# Autodesk Inventor assembly: waterjet assembly version
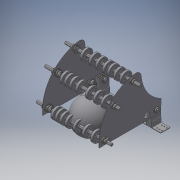
[picture p0: Inventor's stored thumbnail of the model, 180x180]
Saved by Autodesk Inventor 2018 (Build 220112000, 112)
## iProperties
Created: 2020-01-24
Part Number: waterjet assembly version
Document SubType Name: Assembly
Designer: s-2513225
Author: s-2513225
## Documents named in this file (12)
- \\studenthome\students\S-2513225\GitHub\2020CAD\Over bumper intake\Assembly\waterjet assembly version.iam
- \\studenthome\students\S-2513225\GitHub\2020CAD\Over bumper intake\Parts\waterjet wall.ipt
- \\studenthome\students\S-2513225\GitHub\2020CAD\Over bumper intake\Parts\0_500_Hex_ID_x_1_125_OD_x_0_313_WD_Flanged_Bearing_v2_217-3875.ipt
- \\studenthome\students\S-2513225\GitHub\2020CAD\Over bumper intake\Parts\hex shaft 1.ipt
- \\studenthome\students\S-2513225\GitHub\2020CAD\Over bumper intake\Parts\ball mock up.ipt
- \\studenthome\students\S-2513225\GitHub\2020CAD\Over bumper intake\Parts\banebots 400 - 2 3-8 replacement.ipt
- \\studenthome\students\S-2513225\GitHub\2020CAD\Over bumper intake\Parts\anchor point.ipt
- \\studenthome\students\S-2513225\GitHub\2020CAD\Over bumper intake\Parts\hex 2.ipt
- \\studenthome\students\S-2513225\GitHub\2020CAD\Over bumper intake\Parts\2in bracket.ipt
- \\studenthome\students\S-2513225\GitHub\2020CAD\Over bumper intake\Parts\VersaPlanetary_v2_Single_Stage_10_1_with_775_Series.iam
- \\studenthome\students\S-2513225\GitHub\2020CAD\Over bumper intake\Parts\_16t_Aluminum_Hub_Sprocket_25_Chain_1_2_Hex_Bore_217-2642.ipt
- \\studenthome\students\S-2513225\GitHub\2020CAD\Over bumper intake\Parts\Clamping_Shaft_Collar_-_1_2_Hex_ID_217-2737.ipt
## Components (70 placed, 11 different names)
1. waterjet wall:1 — Mate:2, Mate:4, Mate:5, Mate:6, Mate:7, Mate:8, Mate:9, Mate:26, Mate:79, Mate:90, Mate:91, Mate:97, Mate:108, Mate:109, Flush:11, Flush:12, Symmetry:1
2. waterjet wall:2 — Mate:16, Mate:17, Mate:18, Mate:19, Mate:20, Mate:21, Mate:22, Mate:26, Mate:88, Mate:89, Mate:99, Symmetry:1, Flush:13
3. 0_500_Hex_ID_x_1_125_OD_x_0_313_WD_Flanged_Bearing_v2_217-3875:1 — Mate:5, Mate:7, Mate:10, Mate:15
4. 0_500_Hex_ID_x_1_125_OD_x_0_313_WD_Flanged_Bearing_v2_217-3875:2 — Mate:6, Mate:9, Mate:12, Mate:14
5. 0_500_Hex_ID_x_1_125_OD_x_0_313_WD_Flanged_Bearing_v2_217-3875:3 — Mate:4, Mate:8, Mate:11, Mate:13
6. 0_500_Hex_ID_x_1_125_OD_x_0_313_WD_Flanged_Bearing_v2_217-3875:4 — Mate:19, Mate:21, Mate:24
7. 0_500_Hex_ID_x_1_125_OD_x_0_313_WD_Flanged_Bearing_v2_217-3875:5 — Mate:18, Mate:20, Mate:23, Mate:25
8. 0_500_Hex_ID_x_1_125_OD_x_0_313_WD_Flanged_Bearing_v2_217-3875:6 — Mate:17, Mate:22
9. hex shaft 1:1 — Mate:12, Mate:14, Mate:23, Mate:25, Mate:37, Mate:53, Mate:68, Mate:72, Mate:73, Mate:74, Mate:75, Mate:76, Mate:77, Mate:78, Mate:104, Mate:105, Mate:106, Mate:107, Flush:11, Mate:118, Mate:119, Mate:122, Mate:123, Mate:138, Mate:139, Mate:149
10. hex shaft 1:2 — Mate:10, Mate:15, Mate:27, Mate:28, Mate:29, Mate:30, Mate:39, Mate:42, Mate:43, Mate:44, Mate:45, Mate:46, Mate:61, Mate:62, Mate:63, Mate:64, Mate:130, Mate:131, Mate:132, Mate:133, Mate:134, Mate:135, Mate:136, Mate:147
11. hex shaft 1:3 — Mate:11, Mate:13, Mate:24, Mate:31, Mate:32, Mate:33, Mate:34, Mate:40, Mate:47, Mate:48, Mate:49, Mate:50, Mate:51, Mate:65, Mate:66, Mate:69, Mate:70, Mate:124, Mate:125, Mate:126, Mate:127, Mate:128, Mate:129, Mate:137, Mate:148
12. ball mock up:1
13. banebots 400 - 2 3-8 replacement:1 — Mate:27, Mate:42
14. banebots 400 - 2 3-8 replacement:2 — Mate:30, Mate:43
15. banebots 400 - 2 3-8 replacement:3 — Mate:31, Mate:50
16. banebots 400 - 2 3-8 replacement:4 — Mate:29, Mate:44
17. banebots 400 - 2 3-8 replacement:5 — Mate:40, Mate:51
18. banebots 400 - 2 3-8 replacement:6 — Mate:28, Mate:46
19. banebots 400 - 2 3-8 replacement:7 — Mate:34, Mate:47
20. banebots 400 - 2 3-8 replacement:8 — Mate:32, Mate:48
21. banebots 400 - 2 3-8 replacement:9 — Mate:39, Mate:45
22. banebots 400 - 2 3-8 replacement:10 — Mate:73, Mate:78
23. banebots 400 - 2 3-8 replacement:11 — Mate:37, Mate:53
24. banebots 400 - 2 3-8 replacement:12 — Mate:75, Mate:76
25. banebots 400 - 2 3-8 replacement:13 — Mate:105, Mate:106
26. banebots 400 - 2 3-8 replacement:14 — Mate:33, Mate:49
27. banebots 400 - 2 3-8 replacement:15 — Mate:104, Mate:107
28. banebots 400 - 2 3-8 replacement:16 — Mate:61, Mate:63
29. banebots 400 - 2 3-8 replacement:17 — Mate:62, Mate:64
30. banebots 400 - 2 3-8 replacement:18 — Mate:66, Mate:70
31. banebots 400 - 2 3-8 replacement:19 — Mate:65, Mate:69
32. banebots 400 - 2 3-8 replacement:20 — Mate:74, Mate:77
33. banebots 400 - 2 3-8 replacement:21 — Mate:68, Mate:72
34. anchor point:1 — Mate:80, Mate:81, Mate:82, Mate:83, Mate:97, Flush:5, Mate:101, Flush:6, Flush:9, Flush:10, Mate:103
35. anchor point:2 — Mate:84, Mate:85, Mate:86, Mate:87, Mate:99, Mate:100, Flush:3, Flush:4, Mate:102, Flush:7, Flush:8
36. 0_500_Hex_ID_x_1_125_OD_x_0_313_WD_Flanged_Bearing_v2_217-3875:7 — Mate:80, Mate:81, Mate:96
37. 0_500_Hex_ID_x_1_125_OD_x_0_313_WD_Flanged_Bearing_v2_217-3875:8 — Mate:82, Mate:83
38. 0_500_Hex_ID_x_1_125_OD_x_0_313_WD_Flanged_Bearing_v2_217-3875:9 — Mate:84, Mate:85, Mate:98
39. 0_500_Hex_ID_x_1_125_OD_x_0_313_WD_Flanged_Bearing_v2_217-3875:10 — Mate:86, Mate:87
40. 0_500_Hex_ID_x_1_125_OD_x_0_313_WD_Flanged_Bearing_v2_217-3875:11 — Mate:88, Mate:89, Mate:92, Mate:94
41. 0_500_Hex_ID_x_1_125_OD_x_0_313_WD_Flanged_Bearing_v2_217-3875:12 — Mate:90, Mate:91, Mate:93, Mate:95
42. hex 2:1 — Mate:93, Mate:95, Mate:96, Mate:110, Mate:111, Mate:112, Mate:113
43. hex 2:2 — Mate:92, Mate:94, Mate:98, Mate:114, Mate:115, Mate:116, Mate:117
44. 2in bracket:1 — Flush:5, Mate:101, Flush:6, Flush:12
45. 2in bracket:2 — Mate:100, Flush:3, Flush:4, Flush:13
46. 2in bracket:3 — Mate:102, Flush:7, Flush:8
47. 2in bracket:4 — Flush:9, Flush:10, Mate:103
48. VersaPlanetary_v2_Single_Stage_10_1_with_775_Series:1 [sub-assembly] — Mate:142, Mate:143, Mate:144, Mate:145, Mate:146
49. 0_500_Hex_ID_x_1_125_OD_x_0_313_WD_Flanged_Bearing_v2_217-3875:13 — Mate:108, Mate:109, Mate:144
50. _16t_Aluminum_Hub_Sprocket_25_Chain_1_2_Hex_Bore_217-2642:1 — Mate:130, Mate:131
51. _16t_Aluminum_Hub_Sprocket_25_Chain_1_2_Hex_Bore_217-2642:2 — Mate:118, Mate:119
52. _16t_Aluminum_Hub_Sprocket_25_Chain_1_2_Hex_Bore_217-2642:4 — Mate:124, Mate:125
53. Clamping_Shaft_Collar_-_1_2_Hex_ID_217-2737:1 — Mate:122, Mate:123
54. Clamping_Shaft_Collar_-_1_2_Hex_ID_217-2737:2 — Mate:128, Mate:129
55. Clamping_Shaft_Collar_-_1_2_Hex_ID_217-2737:3 — Mate:134, Mate:135
56. Clamping_Shaft_Collar_-_1_2_Hex_ID_217-2737:4 — Mate:138, Mate:139
57. Clamping_Shaft_Collar_-_1_2_Hex_ID_217-2737:5 — Mate:137
58. Clamping_Shaft_Collar_-_1_2_Hex_ID_217-2737:6 — Mate:136
59. Clamping_Shaft_Collar_-_1_2_Hex_ID_217-2737:7 — Mate:114, Mate:115
60. Clamping_Shaft_Collar_-_1_2_Hex_ID_217-2737:8 — Mate:116, Mate:117
61. Clamping_Shaft_Collar_-_1_2_Hex_ID_217-2737:9 — Mate:110, Mate:111
62. Clamping_Shaft_Collar_-_1_2_Hex_ID_217-2737:10 — Mate:112, Mate:113
63. Clamping_Shaft_Collar_-_1_2_Hex_ID_217-2737:11 — Mate:147
64. _16t_Aluminum_Hub_Sprocket_25_Chain_1_2_Hex_Bore_217-2642:5 — Mate:126, Mate:127
65. _16t_Aluminum_Hub_Sprocket_25_Chain_1_2_Hex_Bore_217-2642:6 — Mate:132, Mate:133
66. _16t_Aluminum_Hub_Sprocket_25_Chain_1_2_Hex_Bore_217-2642:7
67. Clamping_Shaft_Collar_-_1_2_Hex_ID_217-2737:12 — Mate:142, Mate:143
68. _16t_Aluminum_Hub_Sprocket_25_Chain_1_2_Hex_Bore_217-2642:8 — Mate:145, Mate:146
69. Clamping_Shaft_Collar_-_1_2_Hex_ID_217-2737:13 — Mate:148
70. Clamping_Shaft_Collar_-_1_2_Hex_ID_217-2737:15 — Mate:149
## Relationships (141: Mate 129, Flush 11, Symmetry 1)
- Mate:2: waterjet wall:1
- Mate:4: waterjet wall:1 ↔ 0_500_Hex_ID_x_1_125_OD_x_0_313_WD_Flanged_Bearing_v2_217-3875:3
- Mate:5: waterjet wall:1 ↔ 0_500_Hex_ID_x_1_125_OD_x_0_313_WD_Flanged_Bearing_v2_217-3875:1
- Mate:6: waterjet wall:1 ↔ 0_500_Hex_ID_x_1_125_OD_x_0_313_WD_Flanged_Bearing_v2_217-3875:2
- Mate:7: waterjet wall:1 ↔ 0_500_Hex_ID_x_1_125_OD_x_0_313_WD_Flanged_Bearing_v2_217-3875:1
- Mate:8: waterjet wall:1 ↔ 0_500_Hex_ID_x_1_125_OD_x_0_313_WD_Flanged_Bearing_v2_217-3875:3
- Mate:9: waterjet wall:1 ↔ 0_500_Hex_ID_x_1_125_OD_x_0_313_WD_Flanged_Bearing_v2_217-3875:2
- Mate:10: 0_500_Hex_ID_x_1_125_OD_x_0_313_WD_Flanged_Bearing_v2_217-3875:1 ↔ hex shaft 1:2
- Mate:11: 0_500_Hex_ID_x_1_125_OD_x_0_313_WD_Flanged_Bearing_v2_217-3875:3 ↔ hex shaft 1:3
- Mate:12: 0_500_Hex_ID_x_1_125_OD_x_0_313_WD_Flanged_Bearing_v2_217-3875:2 ↔ hex shaft 1:1
- Mate:13: 0_500_Hex_ID_x_1_125_OD_x_0_313_WD_Flanged_Bearing_v2_217-3875:3 ↔ hex shaft 1:3
- Mate:14: 0_500_Hex_ID_x_1_125_OD_x_0_313_WD_Flanged_Bearing_v2_217-3875:2 ↔ hex shaft 1:1
- Mate:15: 0_500_Hex_ID_x_1_125_OD_x_0_313_WD_Flanged_Bearing_v2_217-3875:1 ↔ hex shaft 1:2
- Mate:16: waterjet wall:2
- Mate:17: waterjet wall:2 ↔ 0_500_Hex_ID_x_1_125_OD_x_0_313_WD_Flanged_Bearing_v2_217-3875:6
- Mate:18: waterjet wall:2 ↔ 0_500_Hex_ID_x_1_125_OD_x_0_313_WD_Flanged_Bearing_v2_217-3875:5
- Mate:19: waterjet wall:2 ↔ 0_500_Hex_ID_x_1_125_OD_x_0_313_WD_Flanged_Bearing_v2_217-3875:4
- Mate:20: waterjet wall:2 ↔ 0_500_Hex_ID_x_1_125_OD_x_0_313_WD_Flanged_Bearing_v2_217-3875:5
- Mate:21: waterjet wall:2 ↔ 0_500_Hex_ID_x_1_125_OD_x_0_313_WD_Flanged_Bearing_v2_217-3875:4
- Mate:22: waterjet wall:2 ↔ 0_500_Hex_ID_x_1_125_OD_x_0_313_WD_Flanged_Bearing_v2_217-3875:6
- Mate:23: 0_500_Hex_ID_x_1_125_OD_x_0_313_WD_Flanged_Bearing_v2_217-3875:5 ↔ hex shaft 1:1
- Mate:24: 0_500_Hex_ID_x_1_125_OD_x_0_313_WD_Flanged_Bearing_v2_217-3875:4 ↔ hex shaft 1:3
- Mate:25: 0_500_Hex_ID_x_1_125_OD_x_0_313_WD_Flanged_Bearing_v2_217-3875:5 ↔ hex shaft 1:1
- Mate:26 (304.8 mm): waterjet wall:1 ↔ waterjet wall:2
- Mate:27: hex shaft 1:2 ↔ banebots 400 - 2 3-8 replacement:1
- Mate:28: hex shaft 1:2 ↔ banebots 400 - 2 3-8 replacement:6
- Mate:29: hex shaft 1:2 ↔ banebots 400 - 2 3-8 replacement:4
- Mate:30: hex shaft 1:2 ↔ banebots 400 - 2 3-8 replacement:2
- Mate:31: hex shaft 1:3 ↔ banebots 400 - 2 3-8 replacement:3
- Mate:32: hex shaft 1:3 ↔ banebots 400 - 2 3-8 replacement:8
- Mate:33: hex shaft 1:3 ↔ banebots 400 - 2 3-8 replacement:14
- Mate:34: hex shaft 1:3 ↔ banebots 400 - 2 3-8 replacement:7
- Mate:37: hex shaft 1:1 ↔ banebots 400 - 2 3-8 replacement:11
- Mate:39: hex shaft 1:2 ↔ banebots 400 - 2 3-8 replacement:9
- Mate:40: hex shaft 1:3 ↔ banebots 400 - 2 3-8 replacement:5
- Mate:42: hex shaft 1:2 ↔ banebots 400 - 2 3-8 replacement:1
- Mate:43: hex shaft 1:2 ↔ banebots 400 - 2 3-8 replacement:2
- Mate:44: hex shaft 1:2 ↔ banebots 400 - 2 3-8 replacement:4
- Mate:45: hex shaft 1:2 ↔ banebots 400 - 2 3-8 replacement:9
- Mate:46: hex shaft 1:2 ↔ banebots 400 - 2 3-8 replacement:6
- Mate:47: hex shaft 1:3 ↔ banebots 400 - 2 3-8 replacement:7
- Mate:48: hex shaft 1:3 ↔ banebots 400 - 2 3-8 replacement:8
- Mate:49: hex shaft 1:3 ↔ banebots 400 - 2 3-8 replacement:14
- Mate:50: hex shaft 1:3 ↔ banebots 400 - 2 3-8 replacement:3
- Mate:51: hex shaft 1:3 ↔ banebots 400 - 2 3-8 replacement:5
- Mate:53: hex shaft 1:1 ↔ banebots 400 - 2 3-8 replacement:11
- Mate:61: hex shaft 1:2 ↔ banebots 400 - 2 3-8 replacement:16
- Mate:62: hex shaft 1:2 ↔ banebots 400 - 2 3-8 replacement:17
- Mate:63: hex shaft 1:2 ↔ banebots 400 - 2 3-8 replacement:16
- Mate:64: hex shaft 1:2 ↔ banebots 400 - 2 3-8 replacement:17
- Mate:65: hex shaft 1:3 ↔ banebots 400 - 2 3-8 replacement:19
- Mate:66: hex shaft 1:3 ↔ banebots 400 - 2 3-8 replacement:18
- Mate:68: hex shaft 1:1 ↔ banebots 400 - 2 3-8 replacement:21
- Mate:69: hex shaft 1:3 ↔ banebots 400 - 2 3-8 replacement:19
- Mate:70: hex shaft 1:3 ↔ banebots 400 - 2 3-8 replacement:18
- Mate:72: hex shaft 1:1 ↔ banebots 400 - 2 3-8 replacement:21
- Mate:73: hex shaft 1:1 ↔ banebots 400 - 2 3-8 replacement:10
- Mate:74: hex shaft 1:1 ↔ banebots 400 - 2 3-8 replacement:20
- Mate:75: hex shaft 1:1 ↔ banebots 400 - 2 3-8 replacement:12
- Mate:76: hex shaft 1:1 ↔ banebots 400 - 2 3-8 replacement:12
- Mate:77: hex shaft 1:1 ↔ banebots 400 - 2 3-8 replacement:20
- Mate:78: hex shaft 1:1 ↔ banebots 400 - 2 3-8 replacement:10
- Mate:79: waterjet wall:1
- Mate:80: anchor point:1 ↔ 0_500_Hex_ID_x_1_125_OD_x_0_313_WD_Flanged_Bearing_v2_217-3875:7
- Mate:81: anchor point:1 ↔ 0_500_Hex_ID_x_1_125_OD_x_0_313_WD_Flanged_Bearing_v2_217-3875:7
- Mate:82: anchor point:1 ↔ 0_500_Hex_ID_x_1_125_OD_x_0_313_WD_Flanged_Bearing_v2_217-3875:8
- Mate:83: anchor point:1 ↔ 0_500_Hex_ID_x_1_125_OD_x_0_313_WD_Flanged_Bearing_v2_217-3875:8
- Mate:84: anchor point:2 ↔ 0_500_Hex_ID_x_1_125_OD_x_0_313_WD_Flanged_Bearing_v2_217-3875:9
- Mate:85: anchor point:2 ↔ 0_500_Hex_ID_x_1_125_OD_x_0_313_WD_Flanged_Bearing_v2_217-3875:9
- Mate:86: anchor point:2 ↔ 0_500_Hex_ID_x_1_125_OD_x_0_313_WD_Flanged_Bearing_v2_217-3875:10
- Mate:87: anchor point:2 ↔ 0_500_Hex_ID_x_1_125_OD_x_0_313_WD_Flanged_Bearing_v2_217-3875:10
- Mate:88: waterjet wall:2 ↔ 0_500_Hex_ID_x_1_125_OD_x_0_313_WD_Flanged_Bearing_v2_217-3875:11
- Mate:89: waterjet wall:2 ↔ 0_500_Hex_ID_x_1_125_OD_x_0_313_WD_Flanged_Bearing_v2_217-3875:11
- Mate:90: waterjet wall:1 ↔ 0_500_Hex_ID_x_1_125_OD_x_0_313_WD_Flanged_Bearing_v2_217-3875:12
- Mate:91: waterjet wall:1 ↔ 0_500_Hex_ID_x_1_125_OD_x_0_313_WD_Flanged_Bearing_v2_217-3875:12
- Mate:92: 0_500_Hex_ID_x_1_125_OD_x_0_313_WD_Flanged_Bearing_v2_217-3875:11 ↔ hex 2:2
- Mate:93: 0_500_Hex_ID_x_1_125_OD_x_0_313_WD_Flanged_Bearing_v2_217-3875:12 ↔ hex 2:1
- Mate:94: 0_500_Hex_ID_x_1_125_OD_x_0_313_WD_Flanged_Bearing_v2_217-3875:11 ↔ hex 2:2
- Mate:95: 0_500_Hex_ID_x_1_125_OD_x_0_313_WD_Flanged_Bearing_v2_217-3875:12 ↔ hex 2:1
- Mate:96: 0_500_Hex_ID_x_1_125_OD_x_0_313_WD_Flanged_Bearing_v2_217-3875:7 ↔ hex 2:1
- Mate:97: waterjet wall:1 ↔ anchor point:1
- Mate:98: 0_500_Hex_ID_x_1_125_OD_x_0_313_WD_Flanged_Bearing_v2_217-3875:9 ↔ hex 2:2
- Mate:99: waterjet wall:2 ↔ anchor point:2
- Mate:100: anchor point:2 ↔ 2in bracket:2
- Flush:3: anchor point:2 ↔ 2in bracket:2
- Flush:4: anchor point:2 ↔ 2in bracket:2
- Flush:5: anchor point:1 ↔ 2in bracket:1
- Mate:101: anchor point:1 ↔ 2in bracket:1
- Flush:6: anchor point:1 ↔ 2in bracket:1
- Mate:102: anchor point:2 ↔ 2in bracket:3
- Flush:7: anchor point:2 ↔ 2in bracket:3
- Flush:8: anchor point:2 ↔ 2in bracket:3
- Flush:9: anchor point:1 ↔ 2in bracket:4
- Flush:10: anchor point:1 ↔ 2in bracket:4
- Mate:103: anchor point:1 ↔ 2in bracket:4
- Mate:104: hex shaft 1:1 ↔ banebots 400 - 2 3-8 replacement:15
- Mate:105: hex shaft 1:1 ↔ banebots 400 - 2 3-8 replacement:13
- Mate:106: hex shaft 1:1 ↔ banebots 400 - 2 3-8 replacement:13
- Mate:107: hex shaft 1:1 ↔ banebots 400 - 2 3-8 replacement:15
- Mate:108: waterjet wall:1 ↔ 0_500_Hex_ID_x_1_125_OD_x_0_313_WD_Flanged_Bearing_v2_217-3875:13
- Mate:109: waterjet wall:1 ↔ 0_500_Hex_ID_x_1_125_OD_x_0_313_WD_Flanged_Bearing_v2_217-3875:13
- Mate:110 (1.27 mm): hex 2:1 ↔ Clamping_Shaft_Collar_-_1_2_Hex_ID_217-2737:9
- Mate:111 (1.27 mm): hex 2:1 ↔ Clamping_Shaft_Collar_-_1_2_Hex_ID_217-2737:9
- Mate:112 (1.27 mm): hex 2:1 ↔ Clamping_Shaft_Collar_-_1_2_Hex_ID_217-2737:10
- Mate:113 (1.27 mm): hex 2:1 ↔ Clamping_Shaft_Collar_-_1_2_Hex_ID_217-2737:10
- Mate:114 (1.27 mm): hex 2:2 ↔ Clamping_Shaft_Collar_-_1_2_Hex_ID_217-2737:7
- Mate:115 (1.27 mm): hex 2:2 ↔ Clamping_Shaft_Collar_-_1_2_Hex_ID_217-2737:7
- Mate:116 (1.27 mm): hex 2:2 ↔ Clamping_Shaft_Collar_-_1_2_Hex_ID_217-2737:8
- Mate:117 (1.27 mm): hex 2:2 ↔ Clamping_Shaft_Collar_-_1_2_Hex_ID_217-2737:8
- Flush:11 (50.8 mm): waterjet wall:1 ↔ hex shaft 1:1
- Mate:118: hex shaft 1:1 ↔ _16t_Aluminum_Hub_Sprocket_25_Chain_1_2_Hex_Bore_217-2642:2
- Mate:119 (1.27 mm): hex shaft 1:1 ↔ _16t_Aluminum_Hub_Sprocket_25_Chain_1_2_Hex_Bore_217-2642:2
- Mate:122: hex shaft 1:1 ↔ Clamping_Shaft_Collar_-_1_2_Hex_ID_217-2737:1
- Mate:123 (1.27 mm): hex shaft 1:1 ↔ Clamping_Shaft_Collar_-_1_2_Hex_ID_217-2737:1
- Mate:124 (1.27 mm): hex shaft 1:3 ↔ _16t_Aluminum_Hub_Sprocket_25_Chain_1_2_Hex_Bore_217-2642:4
- Mate:125: hex shaft 1:3 ↔ _16t_Aluminum_Hub_Sprocket_25_Chain_1_2_Hex_Bore_217-2642:4
- Mate:126 (1.27 mm): hex shaft 1:3 ↔ _16t_Aluminum_Hub_Sprocket_25_Chain_1_2_Hex_Bore_217-2642:5
- Mate:127: hex shaft 1:3 ↔ _16t_Aluminum_Hub_Sprocket_25_Chain_1_2_Hex_Bore_217-2642:5
- Mate:128 (1.27 mm): hex shaft 1:3 ↔ Clamping_Shaft_Collar_-_1_2_Hex_ID_217-2737:2
- Mate:129: hex shaft 1:3 ↔ Clamping_Shaft_Collar_-_1_2_Hex_ID_217-2737:2
- Mate:130 (1.27 mm): hex shaft 1:2 ↔ _16t_Aluminum_Hub_Sprocket_25_Chain_1_2_Hex_Bore_217-2642:1
- Mate:131: hex shaft 1:2 ↔ _16t_Aluminum_Hub_Sprocket_25_Chain_1_2_Hex_Bore_217-2642:1
- Mate:132 (1.27 mm): hex shaft 1:2 ↔ _16t_Aluminum_Hub_Sprocket_25_Chain_1_2_Hex_Bore_217-2642:6
- Mate:133: hex shaft 1:2 ↔ _16t_Aluminum_Hub_Sprocket_25_Chain_1_2_Hex_Bore_217-2642:6
- Mate:134 (1.27 mm): hex shaft 1:2 ↔ Clamping_Shaft_Collar_-_1_2_Hex_ID_217-2737:3
- Mate:135: hex shaft 1:2 ↔ Clamping_Shaft_Collar_-_1_2_Hex_ID_217-2737:3
- Mate:136 (1.27 mm): hex shaft 1:2 ↔ Clamping_Shaft_Collar_-_1_2_Hex_ID_217-2737:6
- Mate:137 (1.27 mm): hex shaft 1:3 ↔ Clamping_Shaft_Collar_-_1_2_Hex_ID_217-2737:5
- Mate:138 (1.27 mm): hex shaft 1:1 ↔ Clamping_Shaft_Collar_-_1_2_Hex_ID_217-2737:4
- Mate:139: hex shaft 1:1 ↔ Clamping_Shaft_Collar_-_1_2_Hex_ID_217-2737:4
- Mate:142: VersaPlanetary_v2_Single_Stage_10_1_with_775_Series:1 ↔ Clamping_Shaft_Collar_-_1_2_Hex_ID_217-2737:12
- Mate:143: VersaPlanetary_v2_Single_Stage_10_1_with_775_Series:1 ↔ Clamping_Shaft_Collar_-_1_2_Hex_ID_217-2737:12
- Mate:144: VersaPlanetary_v2_Single_Stage_10_1_with_775_Series:1 ↔ 0_500_Hex_ID_x_1_125_OD_x_0_313_WD_Flanged_Bearing_v2_217-3875:13
- Mate:145 (1.27 mm): VersaPlanetary_v2_Single_Stage_10_1_with_775_Series:1 ↔ _16t_Aluminum_Hub_Sprocket_25_Chain_1_2_Hex_Bore_217-2642:8
- Mate:146: VersaPlanetary_v2_Single_Stage_10_1_with_775_Series:1 ↔ _16t_Aluminum_Hub_Sprocket_25_Chain_1_2_Hex_Bore_217-2642:8
- Flush:12 (-48.768 mm): waterjet wall:1 ↔ 2in bracket:1
- Symmetry:1: waterjet wall:1 ↔ waterjet wall:2
- Flush:13 (-48.768 mm): waterjet wall:2 ↔ 2in bracket:2
- Mate:147 (1.27 mm): hex shaft 1:2 ↔ Clamping_Shaft_Collar_-_1_2_Hex_ID_217-2737:11
- Mate:148 (1.27 mm): hex shaft 1:3 ↔ Clamping_Shaft_Collar_-_1_2_Hex_ID_217-2737:13
- Mate:149 (1.27 mm): hex shaft 1:1 ↔ Clamping_Shaft_Collar_-_1_2_Hex_ID_217-2737:15
